# Autodesk Inventor assembly: Joint_3
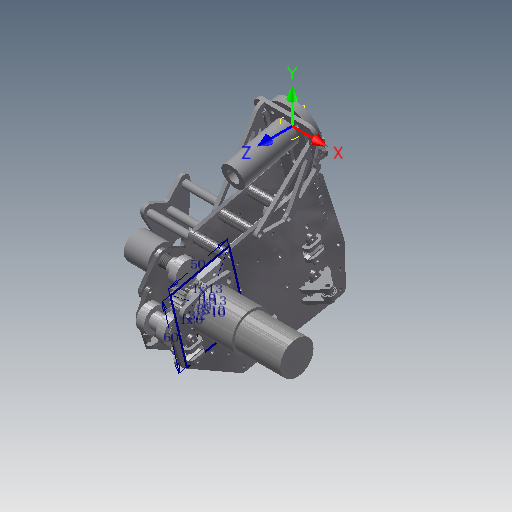
[picture p0: Inventor's stored thumbnail of the model, 512x512]
Saved by Autodesk Inventor 2019.4 (Build 234330000, 330)
## iProperties
Created: 2018-08-09
Part Number: Joint_3
Document SubType Name: Assembly
Designer: Owner
Mass: 579.825 g
Surface Area: 1369.99 cm^2
Volume: 216.499 cm^3
Density: 2.67819 g/cm^3
Author: Owner
## Documents named in this file (27)
- E:\ロボ研\キャチロボ\キャチロボ2019\アーム2019\2019HDarm\Joint_3.iam
- E:\ロボ研\キャチロボ\キャチロボ2019\アーム2019\2019HDarm\ベアリング.ipt
- E:\ロボ研\キャチロボ\キャチロボ2019\アーム2019\2019HDarm\スライダベアリングハウジング.ipt
- E:\ロボ研\キャチロボ\キャチロボ2019\アーム2019\2019HDarm\ラックギア側ベアリング軸.ipt
- E:\ロボ研\キャチロボ\キャチロボ2019\アーム2019\2019HDarm\下側ベアリング軸.ipt
- E:\ロボ研\キャチロボ\キャチロボ2019\アーム2019\2019HDarm\側板ジュラコン.ipt
- E:\ロボ研\キャチロボ\キャチロボ2019\アーム2019\NB_SMF10WW.ipt
- E:\ロボ研\キャチロボ\キャチロボ2019\アーム2019\2019HDarm\2019スライダ側板02.ipt
- E:\ロボ研\キャチロボ\キャチロボ2019\アーム2019\NTN_676A\AIS2019\676A.iam
- E:\ロボ研\キャチロボ\キャチロボ2019\アーム2019\p6l6ALshaft.ipt
- E:\ロボ研\キャチロボ\キャチロボ2019\アーム2019\ShaftBase1.ipt
- E:\ロボ研\キャチロボ\キャチロボ2019\アーム2019\tip.ipt
- E:\ロボ研\キャチロボ\キャチロボ2019\アーム2019\SimLing.ipt
- E:\ロボ研\キャチロボ\キャチロボ2019\アーム2019\NETW5_Autodesk_Inventor_2018_20190615\NETW5.ipt
- E:\ロボ研\キャチロボ\キャチロボ2019\アーム2019\POMベアリング.ipt
- E:\ロボ研\キャチロボ\キャチロボ2019\アーム2019\ShaftBase2.ipt
- E:\ロボ研\キャチロボ\キャチロボ2019\アーム2019\tip2.ipt
- E:\ロボ研\キャチロボ\キャチロボ2019\アーム2019\Tens1.ipt
- E:\ロボ研\キャチロボ\キャチロボ2019\アーム2019\tip3.ipt
- E:\ロボ研\キャチロボ\キャチロボ2019\アーム2019\2019HDarm\Joint_3\デザイン アクセラレータ\平歯車1.iam
- E:\ロボ研\キャチロボ\キャチロボ2019\アーム2019\2019HDarm\RS555-71Mount.ipt
- E:\ロボ研\キャチロボ\キャチロボ2018\アーム\アーム01\RS385PH_Geared_Motor.ipt
- E:\ロボ研\キャチロボ\キャチロボ2018\アーム\アーム01\2axsisSensGear.ipt
- E:\ロボ研\キャチロボ\キャチロボ2018\アーム\ポテンショメータB.ipt
- E:\ロボ研\キャチロボ\キャチロボ2019\アーム2019\2019HDarm\POTplate.ipt
- E:\ロボ研\キャチロボ\キャチロボ2019\アーム2019\2019HDarm\POT2rod.ipt
- E:\ロボ研\キャチロボ\キャチロボ2019\アーム2019\2019HDarm\POT2BASE.ipt
## Components (85 placed, 26 different names)
1. 2019スライダ側板02:1 — 回転:2, 挿入:15, フラッシュ:6, フラッシュ:7, リジッド:11, リジッド:16, リジッド:18, メイト:19, リジッド:37, フラッシュ:8, 回転:15, 回転:16, 回転:17, 回転:18, メイト:21, 回転:21, 回転:22
2. 2019スライダ側板02:2 — リジッド:19, リジッド:27, リジッド:28, 挿入:26, 挿入:32, 挿入:33, 挿入:34, 挿入:35, 挿入:36, リジッド:51, 回転:23, 回転:24, 回転:27, 回転:28, リジッド:60
3. 側板ジュラコン:2 — 挿入:33, 挿入:34
4. スライダベアリングハウジング:1 — リジッド:18, リジッド:19, 回転:13, 回転:14, リジッド:58
5. ラックギア側ベアリング軸:2 — 回転:8, 挿入:35
6. 側板ジュラコン:1 — 回転:2, 挿入:15
7. ベアリング:5 — メイト:6, 挿入:22, メイト:14
8. ベアリング:6 — メイト:7, 挿入:21
9. 下側ベアリング軸:3 — メイト:6, メイト:7, メイト:14, 挿入:26, 挿入:27
10. 676A:1 [sub-assembly] — 回転:4
11. p6l6ALshaft:1 — 回転:4, リジッド:9, リジッド:10
12. ShaftBase1:1 — フラッシュ:6, メイト:10, リジッド:10, リジッド:11
13. ShaftBase1:2 — リジッド:9, フラッシュ:7, メイト:10, リジッド:12
14. tip:1 — リジッド:12
15. 676A:2 [sub-assembly]
16. p6l6ALshaft:2
17. ShaftBase1:3
18. ShaftBase1:4 — リジッド:16
19. tip:2
20. 676A:3 [sub-assembly]
21. p6l6ALshaft:3
22. ShaftBase1:5
23. ShaftBase1:6 — リジッド:28
24. tip:3
25. 676A:4 [sub-assembly]
26. p6l6ALshaft:4
27. ShaftBase1:7
28. ShaftBase1:8 — リジッド:27
29. tip:4
30. SimLing:1 — 挿入:21, 挿入:25
31. SimLing:2 — 挿入:22
32. NETW5:1 — 挿入:25
33. NETW5:2 — 挿入:27
34. ベアリング:7
35. ベアリング:8
36. 下側ベアリング軸:4 — 挿入:32
37. SimLing:3
38. SimLing:4
39. NETW5:3
40. NETW5:4
41. POMベアリング:1 — メイト:19, 回転:8
42. ラックギア側ベアリング軸:3 — 回転:9, 挿入:36
43. POMベアリング:2 — 回転:9
44. NB_SMF10WW:1 — 回転:13, 回転:14
45. Tens1:1 — フラッシュ:8, 回転:15, リジッド:57
46. tip3:1 — リジッド:57
47. tip3:2 — リジッド:59
48. Tens1:2 — リジッド:58, リジッド:59
49. ラックギア側ベアリング軸:4 — 回転:16
50. ラックギア側ベアリング軸:5 — 回転:17
51. ラックギア側ベアリング軸:6 — 回転:18
52. 平歯車:1 [sub-assembly] — メイト:20
53. RS555-71Mount:1 — 挿入:41, 挿入:42, メイト:21, 回転:21, 回転:22
54. RS385PH_Geared_Motor:3 — 挿入:41, 挿入:42, メイト:20
55. 2axsisSensGear:1 — 回転:26
56. POTplate:1 — 回転:23, 回転:24, 回転:25
57. ポテンショメータB:1 — 回転:25, 回転:26
58. POT2rod:1 — 回転:27, 回転:30
59. POT2rod:2 — 回転:28, 回転:29
60. POT2rod:3 — リジッド:60
61. POT2BASE:1 — 回転:29, 回転:30
62. tip2:9 — リジッド:53
63. ShaftBase2:7 — 平面:3, リジッド:53
64. 676A:7 [sub-assembly]
65. p6l6ALshaft:7
66. ShaftBase2:6 — リジッド:51, 平面:3, リジッド:54
67. tip2:5 — リジッド:54
68. ShaftBase2:3 — リジッド:40, 平面:1, リジッド:56
69. p6l6ALshaft:5 — 挿入:37, リジッド:40
70. 676A:5 [sub-assembly]
71. ShaftBase2:1 — リジッド:37, 挿入:37, 平面:1, リジッド:55
72. tip2:1 — リジッド:55
73. tip2:2 — リジッド:56
74. tip2:10
75. ShaftBase2:8
76. 676A:8 [sub-assembly]
77. p6l6ALshaft:8
78. ShaftBase2:9
79. tip2:11
80. ShaftBase2:10
81. p6l6ALshaft:9
82. 676A:9 [sub-assembly]
83. ShaftBase2:11
84. tip2:12
85. tip2:13
## Component patterns: (2 elements, first: tip2:9 + ShaftBase2:7 + 676A:7 + p6l6ALshaft:7 + ShaftBase2:6 + tip2:5 + ShaftBase2:3 + p6l6ALshaft:5 + 676A:5 + ShaftBase2:1 + tip2:1 + tip2:2)
## Relationships (94: WeldJoint 30, RevoluteJoint 25, Insert 19, Mate 15, Flush 3, PlanarJoint 2)
- メイト:6 [Mate]: ベアリング:5 ↔ 下側ベアリング軸:3
- メイト:7 [Mate]: ベアリング:6 ↔ 下側ベアリング軸:3
- [Mate] (-15 mm): ベアリング:5 ↔ ベアリング:6
- 回転:2 [RevoluteJoint]: 2019スライダ側板02:1 ↔ 側板ジュラコン:1
- 挿入:15 [Insert]: 2019スライダ側板02:1 ↔ 側板ジュラコン:1
- 回転:4 [RevoluteJoint]: 676A:1 ↔ p6l6ALshaft:1
- リジッド:9 [WeldJoint]: p6l6ALshaft:1 ↔ ShaftBase1:2
- フラッシュ:6 [Flush]: 2019スライダ側板02:1 ↔ ShaftBase1:1
- フラッシュ:7 [Flush]: 2019スライダ側板02:1 ↔ ShaftBase1:2
- メイト:10 [Mate]: ShaftBase1:1 ↔ ShaftBase1:2
- リジッド:10 [WeldJoint]: p6l6ALshaft:1 ↔ ShaftBase1:1
- リジッド:11 [WeldJoint]: 2019スライダ側板02:1 ↔ ShaftBase1:1
- リジッド:12 [WeldJoint]: ShaftBase1:2 ↔ tip:1
- [RevoluteJoint]: 676A:2 ↔ p6l6ALshaft:2
- [WeldJoint]: p6l6ALshaft:2 ↔ ShaftBase1:4
- [Mate]: ShaftBase1:3 ↔ ShaftBase1:4
- [WeldJoint]: p6l6ALshaft:2 ↔ ShaftBase1:3
- [WeldJoint]: ShaftBase1:4 ↔ tip:2
- リジッド:16 [WeldJoint]: 2019スライダ側板02:1 ↔ ShaftBase1:4
- リジッド:18 [WeldJoint]: 2019スライダ側板02:1 ↔ スライダベアリングハウジング:1
- リジッド:19 [WeldJoint]: 2019スライダ側板02:2 ↔ スライダベアリングハウジング:1
- [RevoluteJoint]: 676A:3 ↔ p6l6ALshaft:3
- [WeldJoint]: p6l6ALshaft:3 ↔ ShaftBase1:6
- [Mate]: ShaftBase1:5 ↔ ShaftBase1:6
- [WeldJoint]: p6l6ALshaft:3 ↔ ShaftBase1:5
- [WeldJoint]: ShaftBase1:6 ↔ tip:3
- [RevoluteJoint]: 676A:4 ↔ p6l6ALshaft:4
- [WeldJoint]: p6l6ALshaft:4 ↔ ShaftBase1:8
- [Mate]: ShaftBase1:7 ↔ ShaftBase1:8
- [WeldJoint]: p6l6ALshaft:4 ↔ ShaftBase1:7
- [WeldJoint]: ShaftBase1:8 ↔ tip:4
- リジッド:27 [WeldJoint]: 2019スライダ側板02:2 ↔ ShaftBase1:8
- リジッド:28 [WeldJoint]: 2019スライダ側板02:2 ↔ ShaftBase1:6
- 挿入:21 [Insert]: ベアリング:6 ↔ SimLing:1
- 挿入:22 [Insert]: ベアリング:5 ↔ SimLing:2
- 挿入:25 [Insert]: SimLing:1 ↔ NETW5:1
- メイト:14 [Mate]: ベアリング:5 ↔ 下側ベアリング軸:3
- 挿入:26 [Insert]: 2019スライダ側板02:2 ↔ 下側ベアリング軸:3
- 挿入:27 [Insert]: 下側ベアリング軸:3 ↔ NETW5:2
- [Mate]: ベアリング:7 ↔ 下側ベアリング軸:4
- [Mate]: ベアリング:8 ↔ 下側ベアリング軸:4
- [Mate] (-15 mm): ベアリング:7 ↔ ベアリング:8
- [Insert]: ベアリング:8 ↔ SimLing:3
- [Insert]: ベアリング:7 ↔ SimLing:4
- [Insert]: SimLing:3 ↔ NETW5:3
- [Mate]: ベアリング:7 ↔ 下側ベアリング軸:4
- [Insert]: 下側ベアリング軸:4 ↔ NETW5:4
- 挿入:32 [Insert]: 2019スライダ側板02:2 ↔ 下側ベアリング軸:4
- メイト:19 [Mate]: 2019スライダ側板02:1 ↔ POMベアリング:1
- 挿入:33 [Insert]: 2019スライダ側板02:2 ↔ 側板ジュラコン:2
- 挿入:34 [Insert]: 2019スライダ側板02:2 ↔ 側板ジュラコン:2
- 回転:8 [RevoluteJoint]: ラックギア側ベアリング軸:2 ↔ POMベアリング:1
- 挿入:35 [Insert]: 2019スライダ側板02:2 ↔ ラックギア側ベアリング軸:2
- 回転:9 [RevoluteJoint]: ラックギア側ベアリング軸:3 ↔ POMベアリング:2
- 挿入:36 [Insert]: 2019スライダ側板02:2 ↔ ラックギア側ベアリング軸:3
- [RevoluteJoint]: p6l6ALshaft:5 ↔ 676A:5
- リジッド:37 [WeldJoint]: 2019スライダ側板02:1 ↔ ShaftBase2:1
- 挿入:37 [Insert]: p6l6ALshaft:5 ↔ ShaftBase2:1
- リジッド:40 [WeldJoint]: ShaftBase2:3 ↔ p6l6ALshaft:5
- [RevoluteJoint]: 676A:7 ↔ p6l6ALshaft:7
- [Insert]: p6l6ALshaft:7 ↔ ShaftBase2:6
- [WeldJoint]: ShaftBase2:7 ↔ p6l6ALshaft:7
- リジッド:51 [WeldJoint]: 2019スライダ側板02:2 ↔ ShaftBase2:6
- 平面:1 [PlanarJoint]: ShaftBase2:3 ↔ ShaftBase2:1
- 平面:3 [PlanarJoint]: ShaftBase2:7 ↔ ShaftBase2:6
- リジッド:53 [WeldJoint]: tip2:9 ↔ ShaftBase2:7
- リジッド:54 [WeldJoint]: ShaftBase2:6 ↔ tip2:5
- リジッド:55 [WeldJoint]: ShaftBase2:1 ↔ tip2:1
- リジッド:56 [WeldJoint]: ShaftBase2:3 ↔ tip2:2
- 回転:13 [RevoluteJoint]: スライダベアリングハウジング:1 ↔ NB_SMF10WW:1
- 回転:14 [RevoluteJoint]: スライダベアリングハウジング:1 ↔ NB_SMF10WW:1
- フラッシュ:8 [Flush]: 2019スライダ側板02:1 ↔ Tens1:1
- 回転:15 [RevoluteJoint]: 2019スライダ側板02:1 ↔ Tens1:1
- リジッド:57 [WeldJoint]: Tens1:1 ↔ tip3:1
- リジッド:58 [WeldJoint]: スライダベアリングハウジング:1 ↔ Tens1:2
- リジッド:59 [WeldJoint]: tip3:2 ↔ Tens1:2
- 回転:16 [RevoluteJoint]: 2019スライダ側板02:1 ↔ ラックギア側ベアリング軸:4
- 回転:17 [RevoluteJoint]: 2019スライダ側板02:1 ↔ ラックギア側ベアリング軸:5
- 回転:18 [RevoluteJoint]: 2019スライダ側板02:1 ↔ ラックギア側ベアリング軸:6
- 挿入:41 [Insert]: RS555-71Mount:1 ↔ RS385PH_Geared_Motor:3
- 挿入:42 [Insert]: RS555-71Mount:1 ↔ RS385PH_Geared_Motor:3
- メイト:20 [Mate]: 平歯車:1 ↔ RS385PH_Geared_Motor:3
- メイト:21 [Mate]: 2019スライダ側板02:1 ↔ RS555-71Mount:1
- 回転:21 [RevoluteJoint]: 2019スライダ側板02:1 ↔ RS555-71Mount:1
- 回転:22 [RevoluteJoint]: 2019スライダ側板02:1 ↔ RS555-71Mount:1
- 回転:23 [RevoluteJoint]: 2019スライダ側板02:2 ↔ POTplate:1
- 回転:24 [RevoluteJoint]: 2019スライダ側板02:2 ↔ POTplate:1
- 回転:25 [RevoluteJoint]: POTplate:1 ↔ ポテンショメータB:1
- 回転:26 [RevoluteJoint] (-1 mm): 2axsisSensGear:1 ↔ ポテンショメータB:1
- 回転:27 [RevoluteJoint]: 2019スライダ側板02:2 ↔ POT2rod:1
- 回転:28 [RevoluteJoint]: 2019スライダ側板02:2 ↔ POT2rod:2
- リジッド:60 [WeldJoint]: 2019スライダ側板02:2 ↔ POT2rod:3
- 回転:29 [RevoluteJoint]: POT2rod:2 ↔ POT2BASE:1
- 回転:30 [RevoluteJoint]: POT2rod:1 ↔ POT2BASE:1
## Named parameters: d26_d24 = -15 mm, d28_d21 = 0 mm, d29_d22 = 0 mm, d64_d52 = -174.796119 deg, d65_d57 = 0 mm, d66_d60 = 0 mm, d67_d61 = 0 mm, d68_d63 = 0 mm, d69_d51 = 0 mm, d78_d64_d52 = 16.954629 deg, d79_d65_d57 = 0 mm, d80_d66_d60 = 0 mm, d81_d67_d61 = 0 mm, d82_d68_d63 = 0 mm, d83_d69_d51 = 0 mm, d84_d64_d52 = 0.637746 deg, d85_d65_d57 = 0 mm, d86_d66_d60 = 0 mm, d87_d67_d61 = 0 mm, d88_d68_d63 = 0 mm, d89_d69_d51 = 0 mm, d100_d96 = 0 mm, d101_d97 = 0 mm, d102_d99 = 0 mm, d103_d92 = 0 mm, d104_d93 = 0 mm, d105_d26_d24 = -15 mm, d106_d28_d21 = 0 mm, d107_d29_d22 = 0 mm, d117_d114 = 0 mm, d118_d115 = 2.855402 deg, d120_d84_d64_d52 = 179.399203 deg, d125_d89_d69_d51 = 0 mm, d171_d142 = 0 mm, d172_d120_d84_d64_d52 = -2.244843 deg, d173_d125_d89_d69_d51 = 0 mm, d174_d135 = 0 mm
